# Autodesk Inventor assembly: SA10_MIR
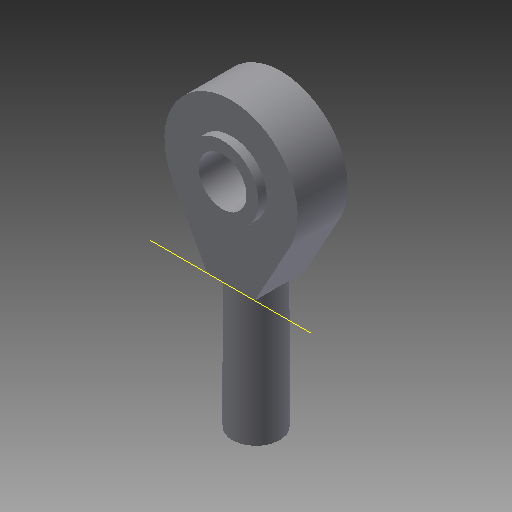
[picture p0: Inventor's stored thumbnail of the model, 512x512]
Saved by Autodesk Inventor 2019 (Build 230136000, 136)
## iProperties
Created: 2019-10-31
Part Number: SA10_MIR
Document SubType Name: Assembly
Designer: Mark
Author: Mark
## Documents named in this file (3)
- C:\Users\Mark\Desktop\7738 Helion Engineering\7738-CAD-prep\Butterfly drive\SA10_MIR.iam
- C:\Users\Mark\Desktop\7738 Helion Engineering\7738-CAD-prep\Butterfly drive\SA10 Bearing_MIR.ipt
- C:\Users\Mark\Desktop\7738 Helion Engineering\7738-CAD-prep\Butterfly drive\SA10T\K_MIR.ipt
## Components (2 placed, 2 different names)
1. SA10 Bearing_MIR:1 — Ball:1
2. K_MIR:1 — Ball:1
## Relationships (1: BallJoint 1)
- Ball:1: SA10 Bearing_MIR:1 ↔ K_MIR:1
